# Autodesk Inventor assembly: Link2
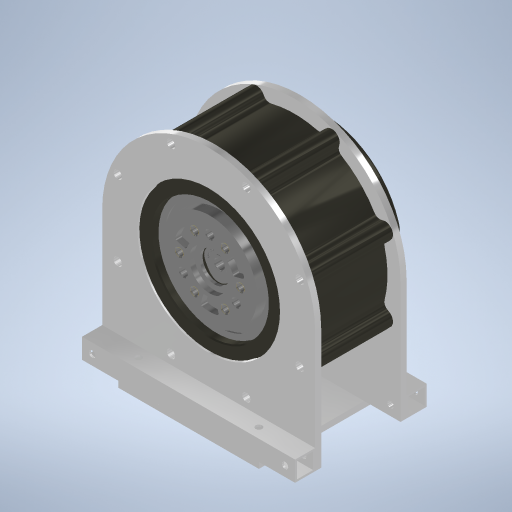
[picture p0: Inventor's stored thumbnail of the model, 512x512]
Saved by Autodesk Inventor 2024 (Build 280153000, 153)
## iProperties
Created: 2024-12-13
Part Number: Link2
Document SubType Name: Assembly
Designer: hirek
Author: hirek
## Documents named in this file (6)
- E:\Documents\Inventor\CanAloha\Link2.iam
- E:\Documents\Inventor\CanAloha\official\robStride03\Robstride03.iam
- E:\Documents\Inventor\CanAloha\myperts\link2_plate1.ipt
- E:\Documents\Inventor\CanAloha\myperts\link2_plate4.ipt
- E:\Documents\Inventor\CanAloha\myperts\link2_plate5.ipt
- E:\Documents\Inventor\CanAloha\myperts\link2_pipe3.ipt
## Components (7 placed, 5 different names)
1. Robstride03:1 [sub-assembly] — 回転:3, 回転:4, 回転:23, 回転:24
2. link2_plate1:1 — 回転:3, 回転:4, 回転:21, 回転:22
3. link2_plate4:1 — 回転:19, 回転:20, 回転:27, 回転:28
4. link2_plate5:1 — 回転:19, 回転:20
5. link2_pipe3:1 — 回転:21, 回転:22, 回転:27
6. link2_plate1:2 — 回転:23, 回転:24, 回転:25, 回転:26
7. link2_pipe3:2 — 回転:25, 回転:26, 回転:28
## Relationships (12: RevoluteJoint 12)
- 回転:3 [RevoluteJoint]: Robstride03:1 ↔ link2_plate1:1
- 回転:4 [RevoluteJoint]: Robstride03:1 ↔ link2_plate1:1
- 回転:19 [RevoluteJoint]: link2_plate4:1 ↔ link2_plate5:1
- 回転:20 [RevoluteJoint]: link2_plate4:1 ↔ link2_plate5:1
- 回転:21 [RevoluteJoint]: link2_plate1:1 ↔ link2_pipe3:1
- 回転:22 [RevoluteJoint]: link2_plate1:1 ↔ link2_pipe3:1
- 回転:23 [RevoluteJoint]: Robstride03:1 ↔ link2_plate1:2
- 回転:24 [RevoluteJoint]: Robstride03:1 ↔ link2_plate1:2
- 回転:25 [RevoluteJoint]: link2_plate1:2 ↔ link2_pipe3:2
- 回転:26 [RevoluteJoint]: link2_plate1:2 ↔ link2_pipe3:2
- 回転:27 [RevoluteJoint]: link2_plate4:1 ↔ link2_pipe3:1
- 回転:28 [RevoluteJoint]: link2_plate4:1 ↔ link2_pipe3:2
